# Autodesk Inventor assembly: Miras
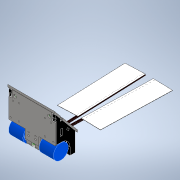
[picture p0: Inventor's stored thumbnail of the model, 180x180]
Saved by Autodesk Inventor 2022 (Build 260153000, 153)
## iProperties
Created: 2022-12-28
Part Number: Miras
Document SubType Name: Assembly
Designer: Kamil
Author: Kamil
## Documents named in this file (22)
- C:\MiniSumo koks\Miras.iam
- C:\MiniSumo koks\blacha_stal_3mm.ipt
- C:\MiniSumo koks\steel_2.ipt
- C:\MiniSumo koks\lead_3.ipt
- C:\MiniSumo koks\Part8.ipt
- C:\MiniSumo koks\n20 motor.ipt
- C:\MiniSumo koks\felga.ipt
- C:\MiniSumo koks\opona.ipt
- C:\MiniSumo koks\strug.ipt
- C:\MiniSumo koks\sciana.ipt
- C:\MiniSumo koks\sciana_MIR.ipt
- C:\MiniSumo koks\mirror.ipt
- C:\MiniSumo koks\uchwyt na plytke.ipt
- C:\MiniSumo koks\wachlarz_1.ipt
- C:\Users\Kamil\Downloads\OLED Display 128x64.ipt
- C:\Users\Kamil\Downloads\pcb_miras_v5.ipt
- C:\MiniSumo koks\montaz_wachlarzy_2.ipt
- C:\MiniSumo koks\wachlarz_1_MIR.ipt
- C:\MiniSumo koks\Serwo_z_widelcem.iam
- C:\MiniSumo koks\widelec.ipt
- C:\MiniSumo koks\PCB_2_Miras.ipt
- C:\Users\Kamil\Downloads\servo horn.ipt
## Components (24 placed, 21 different names)
1. blacha_stal_3mm:1 — Mate:1, Mate:2, Mate:3, Mate:27, Flush:4, Flush:5, Mate:28, Flush:6, Mate:30, Flush:7, Mate:49, Flush:22
2. steel_2:1 — Mate:1, Mate:2, Mate:3, Mate:4, Mate:5, Flush:1
3. lead_3:1 — Mate:4, Mate:5, Flush:1, Flush:2, Flush:3, Mate:16
4. Part8:1 — Flush:2, Flush:3, Mate:11, Mate:12, Mate:13, Mate:14, Mate:15, Mate:18, Mate:37, Flush:9, Flush:10, Flush:14, Mate:55
5. n20 motor:1 — Mate:10, Mate:11, Mate:13, Mate:14, Mate:19, Mate:20, Mate:21
6. n20 motor:2 — Mate:10, Mate:12, Mate:15, Mate:16, Mate:17, Mate:22
7. felga:1 — Mate:17, Mate:18, Mate:22, Mate:24, Mate:25
8. felga:2 — Mate:19, Mate:20, Mate:21, Mate:23, Mate:26
9. opona:1 — Mate:23, Mate:26
10. opona:2 — Mate:24, Mate:25
11. strug:1 — Mate:27, Flush:4, Flush:5, Mate:29, Mate:31, Mate:35, Flush:20, Flush:21, Flush:22
12. sciana:1 — Mate:28, Mate:29, Flush:6, Flush:13, Flush:17, Flush:19
13. sciana_MIR:1 — Mate:30, Flush:7, Mate:31, Flush:8, Mate:36
14. mirror:1 — Mate:35, Flush:8, Mate:36, Flush:21
15. uchwyt na plytke:1 — Mate:37, Flush:9, Flush:10, Mate:44, Flush:15, Mate:50, Mate:51, Mate:58, Flush:18
16. OLED Display 128x64:1 — Mate:44
17. pcb_miras_v5:1 — Mate:49, Flush:13, Flush:14, Flush:17, Flush:19, Flush:20
18. montaz_wachlarzy_2:1 — Flush:15, Mate:50, Mate:51, Mate:52, Mate:53, Mate:54
19. wachlarz_1:2 — Mate:52, Mate:53, Flush:16
20. wachlarz_1_MIR:1 — Mate:54, Flush:16
21. widelec:1 — Mate:55, Mate:56, Mate:57, Mate:60, Mate:61
22. Serwo_z_widelcem:1 [sub-assembly] — Mate:56, Mate:57, Mate:58, Mate:59
23. PCB_2_Miras:1 — Flush:18
24. servo horn:1 — Mate:59, Mate:60, Mate:61
## Relationships (64: Mate 44, Flush 20)
- Mate:1: blacha_stal_3mm:1 ↔ steel_2:1
- Mate:2: blacha_stal_3mm:1 ↔ steel_2:1
- Mate:3: blacha_stal_3mm:1 ↔ steel_2:1
- Mate:4: steel_2:1 ↔ lead_3:1
- Mate:5: steel_2:1 ↔ lead_3:1
- Flush:1: steel_2:1 ↔ lead_3:1
- Flush:2: lead_3:1 ↔ Part8:1
- Flush:3: lead_3:1 ↔ Part8:1
- Mate:10 (5 mm): n20 motor:1 ↔ n20 motor:2
- Mate:11 (2.5 mm): Part8:1 ↔ n20 motor:1
- Mate:12: Part8:1 ↔ n20 motor:2
- Mate:13: Part8:1 ↔ n20 motor:1
- Mate:14: Part8:1 ↔ n20 motor:1
- Mate:15: Part8:1 ↔ n20 motor:2
- Mate:16: lead_3:1 ↔ n20 motor:2
- Mate:17 (0.5 mm): n20 motor:2 ↔ felga:1
- Mate:18: Part8:1 ↔ felga:1
- Mate:19 (0.5 mm): n20 motor:1 ↔ felga:2
- Mate:20: n20 motor:1 ↔ felga:2
- Mate:21: n20 motor:1 ↔ felga:2
- Mate:22: n20 motor:2 ↔ felga:1
- Mate:23: felga:2 ↔ opona:1
- Mate:24: felga:1 ↔ opona:2
- Mate:25: felga:1 ↔ opona:2
- Mate:26: felga:2 ↔ opona:1
- Mate:27: blacha_stal_3mm:1 ↔ strug:1
- Flush:4: blacha_stal_3mm:1 ↔ strug:1
- Flush:5 (2.1 mm): blacha_stal_3mm:1 ↔ strug:1
- Mate:28: blacha_stal_3mm:1 ↔ sciana:1
- Mate:29: strug:1 ↔ sciana:1
- Flush:6: blacha_stal_3mm:1 ↔ sciana:1
- Mate:30: blacha_stal_3mm:1 ↔ sciana_MIR:1
- Flush:7: blacha_stal_3mm:1 ↔ sciana_MIR:1
- Mate:31: strug:1 ↔ sciana_MIR:1
- Mate:35: strug:1 ↔ mirror:1
- Flush:8: sciana_MIR:1 ↔ mirror:1
- Mate:36: sciana_MIR:1 ↔ mirror:1
- Mate:37: Part8:1 ↔ uchwyt na plytke:1
- Flush:9: Part8:1 ↔ uchwyt na plytke:1
- Flush:10: Part8:1 ↔ uchwyt na plytke:1
- Mate:44 (0.4 mm): uchwyt na plytke:1 ↔ OLED Display 128x64:1
- Mate:49 (1.5 mm): blacha_stal_3mm:1 ↔ pcb_miras_v5:1
- Flush:13 (9 mm): sciana:1 ↔ pcb_miras_v5:1
- Flush:14 (1 mm): Part8:1 ↔ pcb_miras_v5:1
- Flush:15: uchwyt na plytke:1 ↔ montaz_wachlarzy_2:1
- Mate:50: uchwyt na plytke:1 ↔ montaz_wachlarzy_2:1
- Mate:51: uchwyt na plytke:1 ↔ montaz_wachlarzy_2:1
- Mate:52: montaz_wachlarzy_2:1 ↔ wachlarz_1:2
- Mate:53: montaz_wachlarzy_2:1 ↔ wachlarz_1:2
- Mate:54: montaz_wachlarzy_2:1 ↔ wachlarz_1_MIR:1
- Flush:16: wachlarz_1:2 ↔ wachlarz_1_MIR:1
- Mate:55: Part8:1 ↔ widelec:1
- Mate:56 (0.5 mm): widelec:1 ↔ Serwo_z_widelcem:1
- Mate:57: widelec:1 ↔ Serwo_z_widelcem:1
- Mate:58: uchwyt na plytke:1 ↔ Serwo_z_widelcem:1
- Flush:17: sciana:1 ↔ pcb_miras_v5:1
- Flush:18: uchwyt na plytke:1 ↔ PCB_2_Miras:1
- Flush:19: sciana:1 ↔ pcb_miras_v5:1
- Flush:20: strug:1 ↔ pcb_miras_v5:1
- Flush:21: strug:1 ↔ mirror:1
- Flush:22: blacha_stal_3mm:1 ↔ strug:1
- Mate:59 (1 mm): Serwo_z_widelcem:1 ↔ servo horn:1
- Mate:60: widelec:1 ↔ servo horn:1
- Mate:61: widelec:1 ↔ servo horn:1
